# Autodesk Inventor assembly: ASY MSC 202 LEFT BOARD
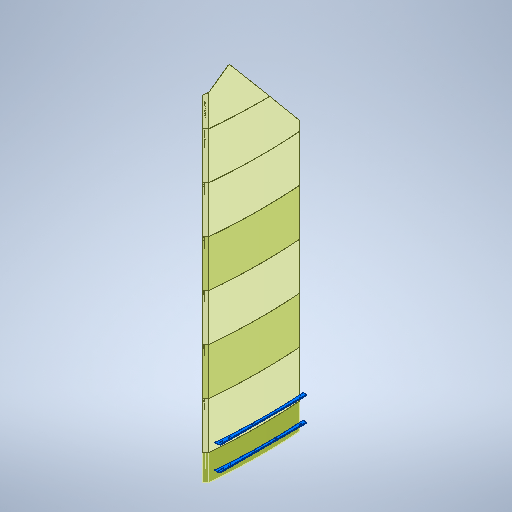
[picture p0: Inventor's stored thumbnail of the model, 512x512]
Saved by Autodesk Inventor 2025 (Build 290162010, 162A)
## iProperties
Created: 2024-07-21
Part Number: ASY MSC 202 LEFT BOARD
Document SubType Name: Assembly
Designer: pokla
Author: pokla
## Documents named in this file (6)
- C:\Users\pokla\Documents\Inventor\Отстойник осветлитель\Manturovo_Se-clar-Gleb\ASY MSC 202 LEFT BOARD.iam
- C:\Users\pokla\Documents\Inventor\Отстойник осветлитель\Manturovo_Se-clar-Gleb\MSC 052 rib board.ipt
- C:\Users\pokla\Documents\Inventor\Отстойник осветлитель\Manturovo_Se-clar-Gleb\MSC 024 sheet board main.ipt
- C:\Users\pokla\Documents\Inventor\Отстойник осветлитель\Manturovo_Se-clar-Gleb\MSC 023 sheet board.ipt
- C:\Users\pokla\Documents\Inventor\Отстойник осветлитель\Manturovo_Se-clar-Gleb\MSC 025 sheet board withers 1.ipt
- C:\Users\pokla\Documents\Inventor\Отстойник осветлитель\Manturovo_Se-clar-Gleb\MSC 027 sheet board face 1.ipt
## Components (10 placed, 5 different names)
1. MSC 052 rib board.ipt:3 — Rigid:16, Flush:4
2. MSC 024 sheet board main.ipt:1 — Rigid:17
3. MSC 024 sheet board main.ipt:2
4. MSC 024 sheet board main.ipt:3
5. MSC 024 sheet board main.ipt:4
6. MSC 024 sheet board main.ipt:5 — Rigid:18
7. MSC 023 sheet board.ipt:1 — Rigid:17, Flush:4
8. MSC 025 sheet board withers 1.ipt:1 — Rigid:18, Rigid:19
9. MSC 027 sheet board face 1.ipt:1 — Rigid:19
10. MSC 052 rib board.ipt:5 — Rigid:16
## Relationships (9: WeldJoint 8, Flush 1)
- [WeldJoint]: MSC 024 sheet board main.ipt:1 ↔ MSC 024 sheet board main.ipt:2
- [WeldJoint]: MSC 024 sheet board main.ipt:2 ↔ MSC 024 sheet board main.ipt:3
- [WeldJoint]: MSC 024 sheet board main.ipt:3 ↔ MSC 024 sheet board main.ipt:4
- [WeldJoint]: MSC 024 sheet board main.ipt:4 ↔ MSC 024 sheet board main.ipt:5
- Rigid:16 [WeldJoint] (-500 mm): MSC 052 rib board.ipt:3 ↔ MSC 052 rib board.ipt:5
- Rigid:17 [WeldJoint]: MSC 024 sheet board main.ipt:1 ↔ MSC 023 sheet board.ipt:1
- Rigid:18 [WeldJoint]: MSC 024 sheet board main.ipt:5 ↔ MSC 025 sheet board withers 1.ipt:1
- Rigid:19 [WeldJoint]: MSC 025 sheet board withers 1.ipt:1 ↔ MSC 027 sheet board face 1.ipt:1
- Flush:4 (304 mm): MSC 052 rib board.ipt:3 ↔ MSC 023 sheet board.ipt:1
